# Autodesk Inventor assembly: hopper assembly
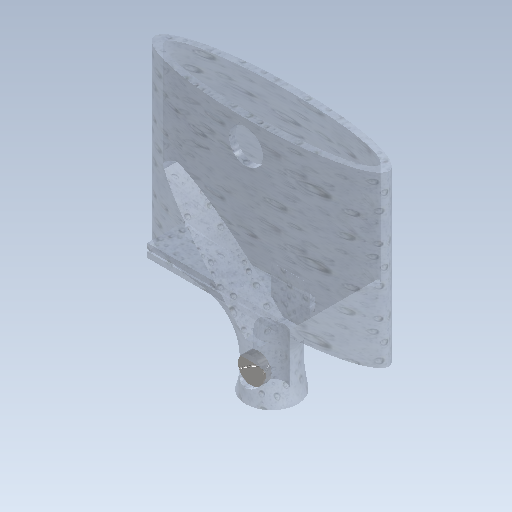
[picture p0: Inventor's stored thumbnail of the model, 512x512]
Saved by Autodesk Inventor 2020 (Build 240168000, 168)
## iProperties
Created: 2021-03-06
Part Number: hopper assembly
Document SubType Name: Assembly
Designer: Harry
Author: Harry
## Documents named in this file (3)
- C:\Users\Harry\Documents\hacktheburgh\octocatch\cad\hopper assembly.iam
- C:\Users\Harry\Documents\hacktheburgh\octocatch\cad\ball hopper.ipt
- C:\Users\Harry\Documents\hacktheburgh\octocatch\cad\electromagnet.ipt
## Components (2 placed, 2 different names)
1. ball hopper:1 — Insert:1
2. electromagnet:1 — Insert:1
## Relationships (1: Insert 1)
- Insert:1 (4 mm): ball hopper:1 ↔ electromagnet:1
